# Autodesk Inventor assembly: EC Sensor Sub-Assem
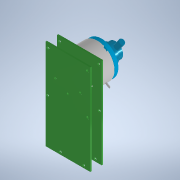
[picture p0: Inventor's stored thumbnail of the model, 180x180]
Saved by Autodesk Inventor 2021 (Build 250183000, 183)
## iProperties
Created: 2020-07-07
Part Number: EC Sensor Sub-Assem
Document SubType Name: Assembly
Designer: jgray
Author: jgray
## Documents named in this file (5)
- M:\Printed Electronics\Gas Sensors\Prototypes\Prototype II -Cartridge Reader V3\EC Sensor Sub-Assem.iam
- M:\Printed Electronics\Gas Sensors\Prototypes\Prototype II -Cartridge Reader V3\EChem Sensor Board Lower.ipt
- M:\Printed Electronics\Gas Sensors\Prototypes\Prototype II -Cartridge Reader V3\EChem Sensor Board.ipt
- M:\Printed Electronics\Gas Sensors\Prototypes\Prototype II -Cartridge Reader V3\S200 EChem Sensor.ipt
- M:\Printed Electronics\Gas Sensors\Prototypes\Prototype II -Cartridge Reader V3\EChem_200 Cap.iam
## Components (4 placed, 4 different names)
1. EChem Sensor Board Lower:1 — Mate:1, Mate:2, Mate:3
2. EChem Sensor Board:1 — Mate:1, Mate:2, Mate:3, Mate:4, Mate:5, Mate:6
3. S200 EChem Sensor:1 — Mate:4, Mate:5, Mate:6, Mate:7, Mate:8
4. EChem_200 Cap:1 [sub-assembly] — Mate:7, Mate:8
## Relationships (8: Mate 8)
- Mate:1 (12 mm): EChem Sensor Board Lower:1 ↔ EChem Sensor Board:1
- Mate:2: EChem Sensor Board Lower:1 ↔ EChem Sensor Board:1
- Mate:3: EChem Sensor Board Lower:1 ↔ EChem Sensor Board:1
- Mate:4: EChem Sensor Board:1 ↔ S200 EChem Sensor:1
- Mate:5: EChem Sensor Board:1 ↔ S200 EChem Sensor:1
- Mate:6: EChem Sensor Board:1 ↔ S200 EChem Sensor:1
- Mate:7: S200 EChem Sensor:1 ↔ EChem_200 Cap:1
- Mate:8: S200 EChem Sensor:1 ↔ EChem_200 Cap:1
